# Autodesk Inventor assembly: Assembly2タミヤダンパー　下
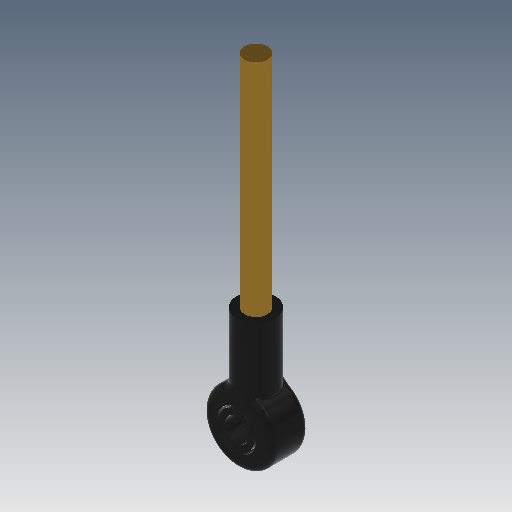
[picture p0: Inventor's stored thumbnail of the model, 512x512]
Saved by Autodesk Inventor 2020.1 (Build 241239000, 239)
## iProperties
Created: 2018-09-18
Part Number: Assembly2タミヤダンパー　下
Material: 一般
Document SubType Name: Assembly
Designer: 杉本　賢二郎
Author: 杉本　賢二郎
## Documents named in this file (4)
- C:\Users\杉本　賢二郎\Desktop\インベンター\新機体制作2020\ダンパー\Assembly2タミヤダンパー_フロント下.iam
- C:\Users\杉本　賢二郎\Desktop\インベンター\新機体制作2020\ダンパー\タミヤダンパー部品7.ipt
- C:\Users\杉本　賢二郎\Desktop\インベンター\新機体制作2020\ダンパー\タミヤダンパー部品8.ipt
- C:\Users\杉本　賢二郎\Desktop\インベンター\新機体制作2020\ダンパー\タミヤダンパー部品5_フロント.ipt
## Components (3 placed, 3 different names)
1. タミヤダンパー部品7:1 — 挿入:1, 挿入:2
2. タミヤダンパー部品8:1 — 挿入:1
3. タミヤダンパー部品5_フロント:1 — 挿入:2
## Relationships (2: Insert 2)
- 挿入:1 [Insert]: タミヤダンパー部品7:1 ↔ タミヤダンパー部品8:1
- 挿入:2 [Insert]: タミヤダンパー部品7:1 ↔ タミヤダンパー部品5_フロント:1
